# Autodesk Inventor assembly: A2017_T3_04
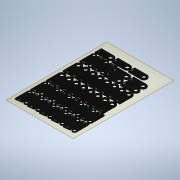
[picture p0: Inventor's stored thumbnail of the model, 180x180]
Saved by Autodesk Inventor 2022 (Build 260153000, 153)
## iProperties
Created: 2022-09-28
Part Number: A2017_T3_04
Document SubType Name: Assembly
Designer: Masato
Author: Masato
## Documents named in this file (4)
- C:\Users\6343y\ドキュメント\Inventor\SUSTAINA-OP\Cam\A2017_T3\A2017_T3_04.iam
- C:\Users\6343y\ドキュメント\Inventor\SUSTAINA-OP\Cam\DisposableBoard.ipt
- C:\Users\6343y\ドキュメント\Inventor\SUSTAINA-OP\LowerBody\Foot\Foot_front_frame.ipt
- C:\Users\6343y\ドキュメント\Inventor\SUSTAINA-OP\LowerBody\Foot\Foot_back_frame.ipt
## Components (48 placed, 3 different names)
1. DisposableBoard:1 — フラッシュ:1, フラッシュ:2, フラッシュ:3, フラッシュ:4, フラッシュ:6, 正接:1, フラッシュ:7, フラッシュ:8, フラッシュ:9
2. Foot_front_frame:1 — メイト:1, フラッシュ:6, メイト:3
3. Foot_front_frame:2 — メイト:2, 正接:1, メイト:3
4. Foot_front_frame:3
5. Foot_front_frame:4 — メイト:5
6. Foot_front_frame:5
7. Foot_front_frame:6
8. Foot_front_frame:7
9. Foot_front_frame:8
10. Foot_front_frame:9
11. Foot_front_frame:10
12. Foot_front_frame:11
13. Foot_front_frame:12
14. Foot_front_frame:13
15. Foot_front_frame:14
16. Foot_front_frame:15
17. Foot_front_frame:16
18. Foot_front_frame:17
19. Foot_front_frame:18
20. Foot_front_frame:19
21. Foot_front_frame:20
22. Foot_back_frame:1 — メイト:4, フラッシュ:7, メイト:5
23. Foot_back_frame:2 — 正接:2
24. Foot_back_frame:3
25. Foot_back_frame:4 — 正接:6
26. Foot_back_frame:5
27. Foot_back_frame:6
28. Foot_back_frame:7
29. Foot_back_frame:8
30. Foot_back_frame:9
31. Foot_back_frame:10 — 正接:5
32. Foot_back_frame:11
33. Foot_back_frame:12
34. Foot_back_frame:13
35. Foot_back_frame:14
36. Foot_back_frame:15
37. Foot_back_frame:16
38. Foot_front_frame:21 — メイト:7, フラッシュ:8, 正接:2, メイト:10, 正接:7
39. Foot_front_frame:22 — メイト:6, メイト:10, 正接:6
40. Foot_front_frame:23
41. Foot_front_frame:24 — メイト:9
42. Foot_back_frame:17 — メイト:8, メイト:9, 正接:5
43. Foot_back_frame:18
44. Foot_back_frame:19
45. Foot_back_frame:20
46. Foot_back_frame:21 — メイト:11, 正接:7, フラッシュ:9
47. Foot_back_frame:22
48. Foot_back_frame:23
## Component patterns: (10 elements, first: Foot_front_frame:1 + Foot_front_frame:2), (16 elements, first: Foot_back_frame:1), (2 elements, first: Foot_front_frame:21 + Foot_front_frame:22), (4 elements, first: Foot_back_frame:17), (3 elements, first: Foot_back_frame:21)
## Relationships (24: Mate 11, Flush 8, Tangent 5)
- フラッシュ:1 [Flush]: DisposableBoard:1
- フラッシュ:2 [Flush]: DisposableBoard:1
- フラッシュ:3 [Flush]: DisposableBoard:1
- フラッシュ:4 [Flush]: DisposableBoard:1
- メイト:1 [Mate]: Foot_front_frame:1
- フラッシュ:6 [Flush] (2.1 mm): DisposableBoard:1 ↔ Foot_front_frame:1
- メイト:2 [Mate]: Foot_front_frame:2
- 正接:1 [Tangent] (2.1 mm): DisposableBoard:1 ↔ Foot_front_frame:2
- メイト:3 [Mate] (2.1 mm): Foot_front_frame:1 ↔ Foot_front_frame:2
- メイト:4 [Mate]: Foot_back_frame:1
- フラッシュ:7 [Flush] (2.1 mm): DisposableBoard:1 ↔ Foot_back_frame:1
- メイト:5 [Mate] (2.1 mm): Foot_front_frame:4 ↔ Foot_back_frame:1
- メイト:6 [Mate]: Foot_front_frame:22
- メイト:7 [Mate]: Foot_front_frame:21
- メイト:8 [Mate]: Foot_back_frame:17
- フラッシュ:8 [Flush] (2.1 mm): DisposableBoard:1 ↔ Foot_front_frame:21
- 正接:2 [Tangent] (3 mm): Foot_back_frame:2 ↔ Foot_front_frame:21
- メイト:9 [Mate] (2.1 mm): Foot_front_frame:24 ↔ Foot_back_frame:17
- 正接:5 [Tangent] (2.1 mm): Foot_back_frame:10 ↔ Foot_back_frame:17
- メイト:10 [Mate] (2.1 mm): Foot_front_frame:21 ↔ Foot_front_frame:22
- 正接:6 [Tangent] (2.1 mm): Foot_back_frame:4 ↔ Foot_front_frame:22
- メイト:11 [Mate]: Foot_back_frame:21
- 正接:7 [Tangent] (2.5 mm): Foot_front_frame:21 ↔ Foot_back_frame:21
- フラッシュ:9 [Flush] (2.1 mm): DisposableBoard:1 ↔ Foot_back_frame:21
